# Autodesk Inventor assembly: Marco_Bicicleta
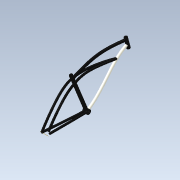
[picture p0: Inventor's stored thumbnail of the model, 180x180]
Saved by Autodesk Inventor 2021 (Build 250183000, 183)
## iProperties
Created: 2021-03-29
Part Number: Marco_Bicicleta
Document SubType Name: Assembly
Designer: j2seb
_SolveAssemblyDoc: Frame Generator Solve Assembly
_Version: 25.0.0
Author: j2seb
## Documents named in this file (3)
- C:\Git\Proyecto_APM\02 Inventor\Marco_Bicicleta.iam
- C:\Git\Proyecto_APM\02 Inventor\Esqueleto_estructura.ipt
- C:\Git\Proyecto_APM\02 Inventor\Marco_Bicicleta\Frame\Estructura 1617045494032.iam
## Components (2 placed, 2 different names)
1. Esqueleto_estructura:1 — Coincidencia:1
2. Estructura 1617045494032:1 [sub-assembly]
## Relationships (2: Mate 1, Angle 1)
- Coincidencia:1 [Mate]: Esqueleto_estructura:1
- Ángulo:1 [Angle] (0 deg)
